# Autodesk Inventor assembly: boron-target-cell
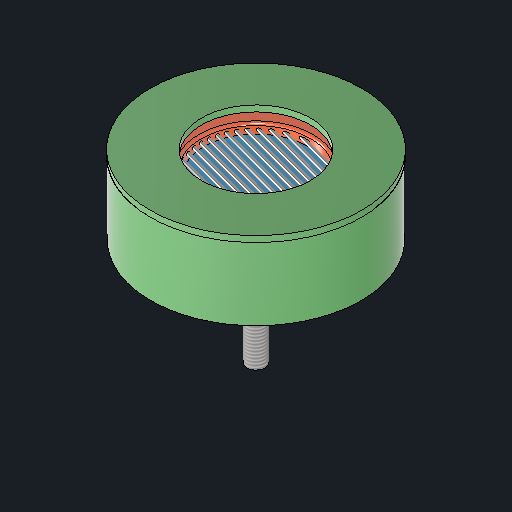
[picture p0: Inventor's stored thumbnail of the model, 512x512]
Saved by Autodesk Inventor 2026 (Build 300175050, 175E)
## iProperties
Created: 2024-10-31
Part Number: boron-target-cell
Document SubType Name: Assembly
Designer: kuzmin
Author: kuzmin
## Documents named in this file (11)
- C:\Users\queez\Dropbox\Drawings\PIHTI\Plasma Vessel\Boron-Target\boron-target-cell.iam
- C:\Users\queez\Dropbox\Drawings\PIHTI\Plasma Vessel\Boron-Target\boron-dish.ipt
- C:\Users\queez\Dropbox\Drawings\PIHTI\Plasma Vessel\Boron-Target\skirt-cylinder.ipt
- C:\Users\queez\Dropbox\Drawings\PIHTI\Plasma Vessel\Boron-Target\skirt-base.ipt
- C:\Users\queez\Dropbox\Drawings\PIHTI\ContentCenter\Ceramics\ceramic_bushing_M3-v1.ipt
- C:\Users\queez\Dropbox\Drawings\PIHTI\ContentCenter\Ceramics\ceramic_washer_M4_v1.ipt
- C:\Users\queez\Dropbox\Drawings\PIHTI\Plasma Vessel\Boron-Target\m3-pin-boron.ipt
- C:\Users\queez\Dropbox\Drawings\PIHTI\ContentCenter\Fastners\M3-nut.ipt
- C:\Users\queez\Dropbox\Drawings\PIHTI\Plasma Vessel\Boron-Target\skirt-lid-for-grooved-targetr.ipt
- C:\Users\queez\Dropbox\Drawings\PIHTI\Plasma Vessel\Boron-Target\mesh.ipt
- C:\Users\queez\Dropbox\Drawings\PIHTI\Plasma Vessel\Boron-Target\boron-under-mesh-plate.ipt
## Components (11 placed, 10 different names)
1. skirt-base:1 — Rigid:2, Rigid:3, Rigid:4, Mate:7, Flush:1, Flush:2
2. boron-dish:1 — Mate:5, Mate:6, Rigid:9, Rigid:10
3. skirt-cylinder:1 — Rigid:2, Rigid:8
4. ceramic_bushing_M3-v1:1 — Rigid:3, Mate:3, Rigid:6
5. ceramic_washer_M4_v1:1 — Rigid:4, Rigid:5
6. m3-pin-boron:1 — Mate:3, Mate:5
7. JIS B 1181 Style 1 - Metric A M3:1 — Rigid:5, Mate:6
8. JIS B 1181 Style 1 - Metric A M3:2 — Rigid:6
9. skirt-lid-for-grooved-targetr:1 — Rigid:8
10. mesh:1 — Rigid:9
11. boron-under-mesh-plate:1 — Rigid:10
## Relationships (15: WeldJoint 8, Mate 5, Flush 2)
- [Mate]: boron-dish:1 ↔ skirt-cylinder:1
- Rigid:2 [WeldJoint]: skirt-base:1 ↔ skirt-cylinder:1
- Rigid:3 [WeldJoint]: skirt-base:1 ↔ ceramic_bushing_M3-v1:1
- Rigid:4 [WeldJoint]: skirt-base:1 ↔ ceramic_washer_M4_v1:1
- Mate:3: ceramic_bushing_M3-v1:1 ↔ m3-pin-boron:1
- Mate:5: boron-dish:1 ↔ m3-pin-boron:1
- Rigid:5 [WeldJoint]: ceramic_washer_M4_v1:1 ↔ JIS B 1181 Style 1 - Metric A M3:1
- Rigid:6 [WeldJoint]: ceramic_bushing_M3-v1:1 ↔ JIS B 1181 Style 1 - Metric A M3:2
- Mate:6: boron-dish:1 ↔ JIS B 1181 Style 1 - Metric A M3:1
- Mate:7: skirt-base:1
- Flush:1: skirt-base:1
- Flush:2: skirt-base:1
- Rigid:8 [WeldJoint]: skirt-cylinder:1 ↔ skirt-lid-for-grooved-targetr:1
- Rigid:9 [WeldJoint]: boron-dish:1 ↔ mesh:1
- Rigid:10 [WeldJoint]: boron-dish:1 ↔ boron-under-mesh-plate:1
